# Autodesk Inventor assembly: B7B9384D898D
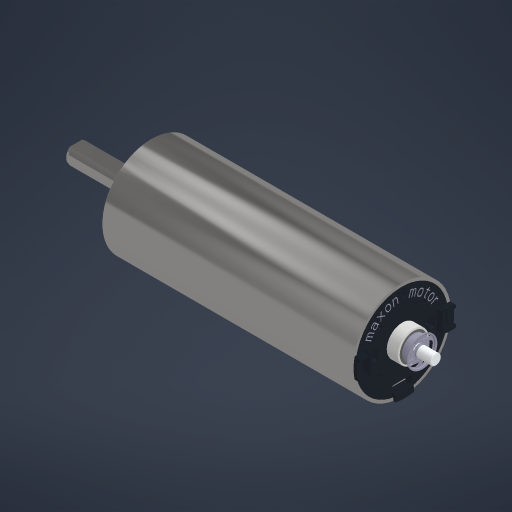
[picture p0: Inventor's stored thumbnail of the model, 512x512]
Saved by Autodesk Inventor 2023 (Build 270158000, 158)
## iProperties
Company: CADClick - www.CADClick.com
Created: 2020-06-14
Part Number: B7B9384D898D
Description: STEP AP214
Document SubType Name: Assembly
Designer: EB
Authority: unknown authorization
Preprocessor: Spatial InterOp 3D
Title: cctmp_9C7EF08E-B654-4BC2-BFD6-390B871BB038_2020_6_14_14_47_32_254..stp
Author: maxon motor ag
Revision Number: NONE
## Documents named in this file (8)
- C:\Users\Elias Braun\Nextcloud2\RoboCup2023\Motor\Maxon\B7B9384D898D.iam
- C:\Users\Elias Braun\Nextcloud2\RoboCup2023\Motor\Maxon\0.ipt
- C:\Users\Elias Braun\Nextcloud2\RoboCup2023\Motor\Maxon\0_1.ipt
- C:\Users\Elias Braun\Nextcloud2\RoboCup2023\Motor\Maxon\0_2.ipt
- C:\Users\Elias Braun\Nextcloud2\RoboCup2023\Motor\Maxon\0_3.ipt
- C:\Users\Elias Braun\Nextcloud2\RoboCup2023\Motor\Maxon\0_4.ipt
- C:\Users\Elias Braun\Nextcloud2\RoboCup2023\Motor\Maxon\0_5.ipt
- C:\Users\Elias Braun\Nextcloud2\RoboCup2023\Motor\Maxon\0_6.ipt
## Components (7 placed, 7 different names)
1. 0 — Mate:1, Mate:2
2. 0_1 — Mate:1, Mate:2, Mate:3, Mate:4
3. 0_2 — Mate:3, Mate:4, Mate:5, Mate:6
4. 0_3
5. 0_4 — Mate:7, Mate:8, Mate:9, Mate:10
6. 0_5 — Mate:9, Mate:10
7. 0_6 — Mate:5, Mate:6, Mate:7, Mate:8
## Relationships (10: Mate 10)
- Mate:1: 0 ↔ 0_1
- Mate:2: 0 ↔ 0_1
- Mate:3: 0_1 ↔ 0_2
- Mate:4 (-1.25 mm): 0_1 ↔ 0_2
- Mate:5: 0_2 ↔ 0_6
- Mate:6: 0_2 ↔ 0_6
- Mate:7: 0_4 ↔ 0_6
- Mate:8: 0_4 ↔ 0_6
- Mate:9: 0_4 ↔ 0_5
- Mate:10: 0_4 ↔ 0_5
